# Autodesk Inventor assembly: 2nd frameiam
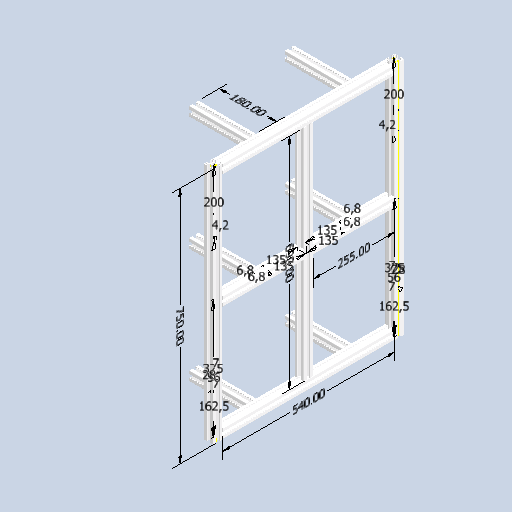
[picture p0: Inventor's stored thumbnail of the model, 512x512]
Saved by Autodesk Inventor 2023 (Build 270158000, 158)
## iProperties
Created: 2023-09-03
Part Number: 2nd frameiam
Document SubType Name: Assembly
Designer: sigit
Author: sigit
## Documents named in this file (6)
- D:\Kuliah\SEMESTER 7\Robot Semprot\Design\REVISI2\Assembly\2nd frameiam.iam
- D:\Kuliah\SEMESTER 7\Robot Semprot\Design\REVISI2\Part\tslot 3030 750mm.ipt
- D:\Kuliah\SEMESTER 7\Robot Semprot\Design\REVISI2\Part\tslot 3030 540mm.ipt
- D:\Kuliah\SEMESTER 7\Robot Semprot\Design\REVISI2\Part\tslot 3030 690mm.ipt
- D:\Kuliah\SEMESTER 7\Robot Semprot\Design\REVISI2\Part\tslot 3030 255mm.ipt
- D:\Kuliah\SEMESTER 7\Robot Semprot\Design\REVISI2\Part\tslot 3030 180mm.ipt
## Components (13 placed, 5 different names)
1. tslot 3030 750mm:1 — Rotational:2, Rotational:3
2. tslot 3030 750mm:2 — Rotational:1, Rotational:5
3. tslot 3030 540mm:1 — Rotational:1, Rotational:2, Rigid:2
4. tslot 3030 540mm:2 — Rotational:3, Rotational:4
5. tslot 3030 690mm:1 — Rotational:4, Rotational:6
6. tslot 3030 255mm:2 — Rotational:5, Rotational:7
7. tslot 3030 180mm:1 — Rigid:1
8. tslot 3030 180mm:2 — Rotational:7
9. tslot 3030 255mm:3 — Rotational:6, Rigid:1
10. tslot 3030 180mm:3 — Rigid:2
11. tslot 3030 180mm:4
12. tslot 3030 180mm:5
13. tslot 3030 180mm:6
## Component patterns: (2 elements), (2 elements, first: tslot 3030 180mm:3), Component Pattern 1:2 (2 elements)
## Relationships (9: RevoluteJoint 7, WeldJoint 2)
- Rotational:1 [RevoluteJoint] (-9.486 mm): tslot 3030 750mm:2 ↔ tslot 3030 540mm:1
- Rotational:2 [RevoluteJoint] (9.486 mm): tslot 3030 750mm:1 ↔ tslot 3030 540mm:1
- Rotational:3 [RevoluteJoint] (-9.486 mm): tslot 3030 750mm:1 ↔ tslot 3030 540mm:2
- Rotational:4 [RevoluteJoint] (-9.486 mm): tslot 3030 540mm:2 ↔ tslot 3030 690mm:1
- Rotational:5 [RevoluteJoint] (-9.486 mm): tslot 3030 750mm:2 ↔ tslot 3030 255mm:2
- Rotational:6 [RevoluteJoint] (-9.486 mm): tslot 3030 690mm:1 ↔ tslot 3030 255mm:3
- Rigid:1 [WeldJoint] (9.486 mm): tslot 3030 180mm:1 ↔ tslot 3030 255mm:3
- Rotational:7 [RevoluteJoint] (9.486 mm): tslot 3030 255mm:2 ↔ tslot 3030 180mm:2
- Rigid:2 [WeldJoint] (-9.486 mm): tslot 3030 540mm:1 ↔ tslot 3030 180mm:3
